# Autodesk Inventor assembly: CatFeeder
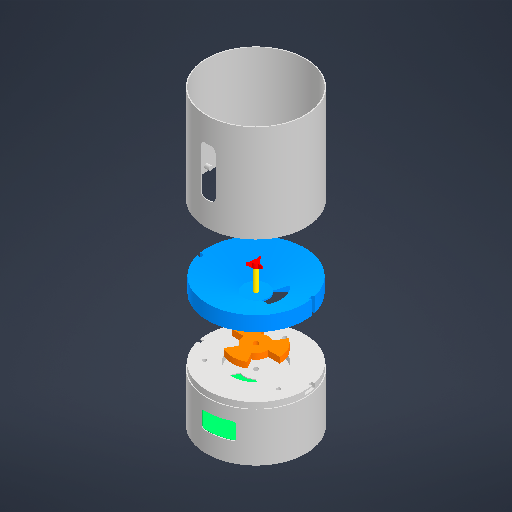
[picture p0: Inventor's stored thumbnail of the model, 512x512]
Saved by Autodesk Inventor 2025.1 (Build 291241020, 241B)
## iProperties
Created: 2024-09-16
Part Number: CatFeeder
Document SubType Name: Assembly
Designer: maxim
Author: maxim
## Documents named in this file (8)
- C:\Users\maxim\OneDrive - Linköpings universitet\Documents\Autodesk\Inventor\CatFeeder2\CatFeeder.iam
- C:\Users\maxim\OneDrive - Linköpings universitet\Documents\Autodesk\Inventor\CatFeeder2\base.ipt
- C:\Users\maxim\OneDrive - Linköpings universitet\Documents\Autodesk\Inventor\CatFeeder2\rotor.ipt
- C:\Users\maxim\OneDrive - Linköpings universitet\Documents\Autodesk\Inventor\CatFeeder2\feeder.ipt
- C:\Users\maxim\OneDrive - Linköpings universitet\Documents\Autodesk\Inventor\CatFeeder2\tube.ipt
- C:\Users\maxim\OneDrive - Linköpings universitet\Documents\Autodesk\Inventor\CatFeeder2\shaft.ipt
- C:\Users\maxim\OneDrive - Linköpings universitet\Documents\Autodesk\Inventor\CatFeeder2\cover.ipt
- C:\Users\maxim\OneDrive - Linköpings universitet\Documents\Autodesk\Inventor\CatFeeder2\cap.ipt
## Components (7 placed, 7 different names)
1. base:1 — Mate:1, Mate:6, Mate:9, Mate:10, Flush:1, Flush:2, Mate:13
2. rotor:1 — Mate:1, Mate:3, Mate:8
3. feeder:1 — Mate:3, Flush:1
4. tube:1 — Mate:6, Flush:2, Mate:13
5. shaft:1 — Mate:8, Mate:11, Mate:12
6. cover:1 — Mate:9
7. cap:1 — Mate:11, Mate:12
## Relationships (11: Mate 9, Flush 2)
- Mate:1: base:1 ↔ rotor:1
- Mate:3: rotor:1 ↔ feeder:1
- Mate:6: base:1 ↔ tube:1
- Mate:8: rotor:1 ↔ shaft:1
- Mate:9: base:1 ↔ cover:1
- Mate:10: base:1
- Mate:11: shaft:1 ↔ cap:1
- Mate:12: shaft:1 ↔ cap:1
- Flush:1: base:1 ↔ feeder:1
- Flush:2: base:1 ↔ tube:1
- Mate:13: base:1 ↔ tube:1
